# Autodesk Inventor assembly: assem_finger_thumb_linact_v2
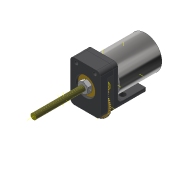
[picture p0: Inventor's stored thumbnail of the model, 180x180]
Saved by Autodesk Inventor 2014 (Build 180170000, 170)
## iProperties
Created: 2015-05-22
Part Number: assem_finger_thumb_linact_v2
Document SubType Name: Assembly
Designer: Martin
Author: Martin
## Documents named in this file (9)
- C:\Users\Martin\Dropbox\biohand-mec\biohand_v1\palm\assem_palm_linact_v2.iam
- C:\Users\Martin\Dropbox\biohand-mec\biohand_v1\palm\linact_palm_cage.ipt
- C:\Users\Martin\Dropbox\biohand-mec\biohand_v1\misc\motor_servo.ipt
- C:\Users\Martin\Dropbox\biohand-mec\biohand_v1\misc\servo_gear_1.ipt
- C:\Users\Martin\Dropbox\biohand-mec\biohand_v1\misc\m2_4_screw.ipt
- C:\Users\Martin\Dropbox\biohand-mec\biohand_v1\palm\linact_palm_front.ipt
- C:\Users\Martin\Dropbox\biohand-mec\biohand_v1\misc\servo_gear_2.ipt
- C:\Users\Martin\Dropbox\biohand-mec\biohand_v1\misc\m3_30_screw.ipt
- C:\Users\Martin\Dropbox\biohand-mec\biohand_v1\misc\m3_nut.ipt
## Components (9 placed, 8 different names)
1. linact_palm_cage:1 — Insert:1, Mate:1, Flush:1, Insert:2, Insert:3, Insert:4
2. motor_servo:1 — Insert:1, Mate:1
3. m2_4_screw:1 — Insert:2
4. m2_4_screw:2 — Insert:3
5. servo_gear_1:1 — Insert:4
6. linact_palm_front:1 — Flush:2, Insert:5
7. servo_gear_2:1 — Insert:5, Insert:6, Insert:7
8. m3_30_screw:1 — Insert:6
9. m3_nut:1 — Insert:7
## Relationships (10: Insert 7, Flush 2, Mate 1)
- Insert:1: linact_palm_cage:1 ↔ motor_servo:1
- Mate:1: linact_palm_cage:1 ↔ motor_servo:1
- Flush:1 (2.8 mm): linact_palm_cage:1
- Insert:2: linact_palm_cage:1 ↔ m2_4_screw:1
- Insert:3: linact_palm_cage:1 ↔ m2_4_screw:2
- Insert:4 (0.5 mm): linact_palm_cage:1 ↔ servo_gear_1:1
- Flush:2: linact_palm_front:1
- Insert:5 (0.25 mm): linact_palm_front:1 ↔ servo_gear_2:1
- Insert:6: servo_gear_2:1 ↔ m3_30_screw:1
- Insert:7: servo_gear_2:1 ↔ m3_nut:1
